# Autodesk Inventor assembly: full case
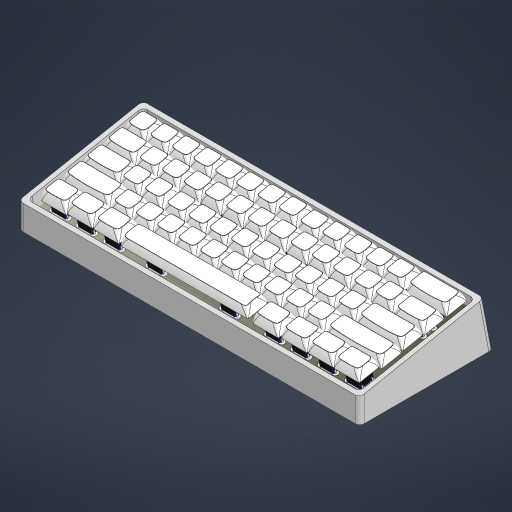
[picture p0: Inventor's stored thumbnail of the model, 512x512]
Saved by Autodesk Inventor 2024.2 (Build 282272000, 272)
## iProperties
Created: 2024-12-04
Part Number: full case
Document SubType Name: Assembly
Designer: Moe
Author: Moe
## Documents named in this file (12)
- D:\Code\git\tiny-keeb\case\full case.iam
- D:\Code\git\tiny-keeb\case\housing.ipt
- D:\Code\git\tiny-keeb\case\references\Raspberry Pi Pico-R3.ipt
- D:\Code\git\tiny-keeb\case\pcb fill in\pcb.ipt
- D:\Code\git\tiny-keeb\caps\cap ref\1u.ipt
- D:\Code\git\tiny-keeb\caps\cap ref\1.5u.ipt
- D:\Code\git\tiny-keeb\caps\cap ref\2u.ipt
- D:\Code\git\tiny-keeb\caps\cap ref\2.25u.ipt
- D:\Code\git\tiny-keeb\caps\cap ref\1.75u.ipt
- D:\Code\git\tiny-keeb\caps\cap ref\1.25u.ipt
- D:\Code\git\tiny-keeb\caps\cap ref\2.75u2.ipt
- D:\Code\git\tiny-keeb\caps\cap ref\6.25u.ipt
## Components (64 placed, 11 different names)
1. housing:1 — Mate:1, Mate:2
2. Raspberry Pi Pico-R3:1
3. pcb:1 — Mate:1, Mate:2, Mate:3, Mate:4, Mate:5, Mate:6, Mate:7, Mate:8, Mate:9, Mate:10, Mate:11, Mate:12, Mate:13, Mate:14, Mate:17, Mate:18, Mate:19
4. 1u:1 — Mate:3
5. 1u:2 — Mate:4
6. 1u:3
7. 1u:4
8. 1u:5
9. 1u:6
10. 1u:7
11. 1u:8
12. 1u:9
13. 1u:10
14. 1u:11
15. 1u:12
16. 1u:13
17. 1u:14
18. 1u:15
19. 1u:16
20. 1u:17
21. 1u:18
22. 1u:19
23. 1u:20
24. 1u:21
25. 1u:22 — Mate:7
26. 1u:23
27. 1u:24 — Mate:5
28. 1u:25 — Mate:6
29. 1u:26
30. 1u:27
31. 1u:28 — Mate:8
32. 1u:29
33. 1u:30
34. 1u:31
35. 1u:32
36. 1u:33
37. 1u:34
38. 1u:35
39. 1u:36
40. 1u:37
41. 1u:38
42. 1u:45
43. 1u:46
44. 1u:47
45. 1u:48
46. 1u:49
47. 1u:51
48. 1u:52
49. 1u:53
50. 1.5u:1 — Mate:9
51. 1.5u:2 — Mate:10
52. 2u:1 — Mate:11
53. 2.25u:1 — Mate:12
54. 1.75u:1 — Mate:13
55. 2.25u:2 — Mate:14
56. 1.25u:1 — Mate:17
57. 1.25u:2
58. 1.25u:3
59. 1.25u:4
60. 1.25u:5
61. 1.25u:6
62. 1.25u:7
63. 2.75u2:1 — Mate:18
64. 6.25u:1 — Mate:19
## Relationships (17: Mate 17)
- Mate:1: housing:1 ↔ pcb:1
- Mate:2: housing:1 ↔ pcb:1
- Mate:3: pcb:1 ↔ 1u:1
- Mate:4: pcb:1 ↔ 1u:2
- Mate:5: pcb:1 ↔ 1u:24
- Mate:6: pcb:1 ↔ 1u:25
- Mate:7: pcb:1 ↔ 1u:22
- Mate:8: pcb:1 ↔ 1u:28
- Mate:9: pcb:1 ↔ 1.5u:1
- Mate:10: pcb:1 ↔ 1.5u:2
- Mate:11: pcb:1 ↔ 2u:1
- Mate:12: pcb:1 ↔ 2.25u:1
- Mate:13: pcb:1 ↔ 1.75u:1
- Mate:14: pcb:1 ↔ 2.25u:2
- Mate:17: pcb:1 ↔ 1.25u:1
- Mate:18: pcb:1 ↔ 2.75u2:1
- Mate:19: pcb:1 ↔ 6.25u:1
